# Autodesk Inventor assembly: LCD-01
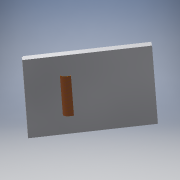
[picture p0: Inventor's stored thumbnail of the model, 180x180]
Saved by Autodesk Inventor 2017 (Build 210142000, 142)
## iProperties
Created: 2018-07-06
Part Number: LCD-01
Document SubType Name: Assembly
Designer: intelsath
Author: intelsath
## Documents named in this file (3)
- C:\Users\intelsath\Documents\Inventor\Cryptowallet\LCD.iam
- C:\Users\intelsath\Documents\Inventor\Cryptowallet\LCD-cable.ipt
- C:\Users\intelsath\Documents\Inventor\Cryptowallet\LCD.ipt
## Components (2 placed, 2 different names)
1. LCD-cable:1 — Flush:2, Mate:1, Mate:2
2. LCD:1 — Flush:2, Mate:1, Mate:2
## Relationships (3: Mate 2, Flush 1)
- Flush:2 (12.35 mm): LCD-cable:1 ↔ LCD:1
- Mate:1 (1.5 mm): LCD-cable:1 ↔ LCD:1
- Mate:2 (-25 mm): LCD-cable:1 ↔ LCD:1
